# Autodesk Inventor assembly: Clutch Assembly
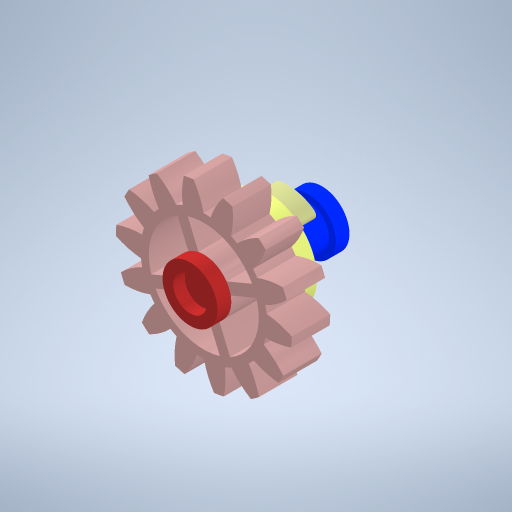
[picture p0: Inventor's stored thumbnail of the model, 512x512]
Saved by Autodesk Inventor 2024.3 (Build 283343000, 343)
## iProperties
Created: 2024-11-08
Part Number: Clutch Assembly
Document SubType Name: Assembly
Designer: wszaf
Author: wszaf
## Documents named in this file (6)
- C:\Users\wszaf\Desktop\Pulpit\3D Printing\Test Prints\Gear Module\Modeling\Clutch\Clutch Assembly.iam
- C:\Users\wszaf\Desktop\Pulpit\3D Printing\Test Prints\Gear Module\Modeling\Gear Related\Gear Assembly\Design Accelerator\Spur Gear12.ipt
- C:\Users\wszaf\Desktop\Pulpit\3D Printing\Test Prints\Gear Module\Print Files\Multiboard Thread insert\Mount Hole Insert\Mount Hole Insert.ipt
- C:\Users\wszaf\Desktop\Pulpit\3D Printing\Test Prints\Gear Module\Print Files\Multiboard Thread insert\Mount Pin Insert\Mount Pin Insert.ipt
- C:\Users\wszaf\Desktop\Pulpit\3D Printing\Test Prints\Gear Module\Modeling\Clutch\Loose Clutch.ipt
- C:\Users\wszaf\Desktop\Pulpit\3D Printing\Test Prints\Gear Module\Modeling\Clutch\Clutch_Pin.ipt
## Components (8 placed, 5 different names)
1. Spur Gear1:1 — Mate:1, Mate:2, Mate:3, Mate:4
2. Spur Gear1:2 — Mate:5, Mate:6, Mate:7, Mate:8, Mate:9, Mate:12
3. Mount Hole Insert:1 — Mate:6, Mate:8
4. Mount Pin Insert:1 — Mate:7, Mate:9, Mate:10
5. Mount Pin Insert:2 — Mate:2, Mate:3
6. Mount Hole Insert:2 — Mate:1, Mate:4, Mate:5, Mate:10, Mate:11
7. Loose Clutch:1 — Mate:11, Mate:12, Flush:1
8. Clutch_Pin:1 — Flush:1
## Relationships (13: Mate 12, Flush 1)
- Mate:1: Spur Gear1:1 ↔ Mount Hole Insert:2
- Mate:2: Spur Gear1:1 ↔ Mount Pin Insert:2
- Mate:3: Spur Gear1:1 ↔ Mount Pin Insert:2
- Mate:4: Spur Gear1:1 ↔ Mount Hole Insert:2
- Mate:5: Spur Gear1:2 ↔ Mount Hole Insert:2
- Mate:6: Spur Gear1:2 ↔ Mount Hole Insert:1
- Mate:7: Spur Gear1:2 ↔ Mount Pin Insert:1
- Mate:8: Spur Gear1:2 ↔ Mount Hole Insert:1
- Mate:9: Spur Gear1:2 ↔ Mount Pin Insert:1
- Mate:10: Mount Pin Insert:1 ↔ Mount Hole Insert:2
- Mate:11: Mount Hole Insert:2 ↔ Loose Clutch:1
- Mate:12: Spur Gear1:2 ↔ Loose Clutch:1
- Flush:1 (-8 mm): Loose Clutch:1 ↔ Clutch_Pin:1
